# Autodesk Inventor assembly: wheelsys
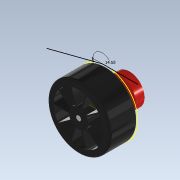
[picture p0: Inventor's stored thumbnail of the model, 180x180]
Saved by Autodesk Inventor 2022 (Build 260153000, 153)
## iProperties
Created: 2023-05-04
Part Number: wheelsys
Document SubType Name: Assembly
Designer: Johnny Jou
Author: Johnny Jou
## Documents named in this file (7)
- C:\Users\Johnny Jou\Documents\GitHub\Areo_Rider_Cabin\car\wheelsys.iam
- C:\Users\Johnny Jou\Documents\GitHub\Areo_Rider_Cabin\car\wheel.ipt
- C:\Users\Johnny Jou\Documents\GitHub\Areo_Rider_Cabin\car\Coupling_0504.ipt
- C:\Users\Johnny Jou\Documents\GitHub\Areo_Rider_Cabin\car\2GT_36T.ipt
- C:\Users\Johnny Jou\Documents\GitHub\Areo_Rider_Cabin\car\axle 4_20.ipt
- C:\Users\Johnny Jou\Documents\GitHub\Areo_Rider_Cabin\car\bearing.ipt
- C:\Users\Johnny Jou\Documents\GitHub\Areo_Rider_Cabin\car\wheel_base_cover.ipt
## Components (7 placed, 6 different names)
1. wheel:1
2. Coupling_0504:1
3. 2GT_36T:1
4. 2GT_36T:2
5. axle 4_20:1
6. 軸承 GB/T 292-2007 類型 IN - 退回 B724 C:1
7. wheel_base_cover:1
## Relationships (14: Mate 13, Flush 1)
- [Mate]: wheel:1 ↔ Coupling_0504:1
- [Mate]: wheel:1 ↔ Coupling_0504:1
- [Mate]: Coupling_0504:1 ↔ 2GT_36T:1
- [Mate]: Coupling_0504:1 ↔ 2GT_36T:1
- [Mate]: Coupling_0504:1 ↔ 2GT_36T:1
- [Mate]: Coupling_0504:1 ↔ 2GT_36T:2
- [Mate]: Coupling_0504:1 ↔ 2GT_36T:2
- [Mate]: 2GT_36T:1 ↔ 2GT_36T:2
- [Mate]: Coupling_0504:1 ↔ axle 4_20:1
- [Mate]: 軸承 GB/T 292-2007 類型 IN - 退回 B724 C:1 ↔ wheel_base_cover:1
- [Mate]: 軸承 GB/T 292-2007 類型 IN - 退回 B724 C:1 ↔ wheel_base_cover:1
- [Mate]: axle 4_20:1 ↔ 軸承 GB/T 292-2007 類型 IN - 退回 B724 C:1
- [Flush]: axle 4_20:1 ↔ 軸承 GB/T 292-2007 類型 IN - 退回 B724 C:1
- [Mate] (5 mm): 2GT_36T:2 ↔ wheel_base_cover:1
## Named parameters: d238_d98 = 0 mm, d239_d99 = 0 mm, d240_d100 = 0 mm, d241_d101 = 0 mm, d242_d102 = 0 mm, d243_d103 = 0 mm, d244_d104 = 0 mm, d245_d105 = 0 mm, d246_d106 = 0 mm, d247_d107 = 0 mm, d248_d108 = 0 mm, d249_d109 = 0 mm, d250_d110 = 0 mm, d251_d111 = 5 mm
